# Autodesk Inventor assembly: Test Assembly
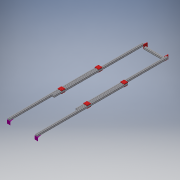
[picture p0: Inventor's stored thumbnail of the model, 180x180]
Saved by Autodesk Inventor 2016 SP2 (Build 200236200, 236)
## iProperties
Created: 2018-01-27
Part Number: Test Assembly
Document SubType Name: Assembly
Designer: CAD
Author: CAD
## Documents named in this file (5)
- C:\Users\CAD\Documents\GitHub\FIRST-ROBOTICS-2018-5436-CAD\Robot\Elevator\Test Assembly.iam
- C:\Users\CAD\Documents\GitHub\FIRST-ROBOTICS-2018-5436-CAD\Robot\Elevator\48 in 80-20 extrusion.ipt
- C:\Users\CAD\Documents\GitHub\FIRST-ROBOTICS-2018-5436-CAD\Robot\Elevator\80-20 extrusion rail.ipt
- C:\Users\CAD\Documents\GitHub\FIRST-ROBOTICS-2018-5436-CAD\Robot\Elevator\Bottom Elevator Bracket.ipt
- C:\Users\CAD\Documents\GitHub\FIRST-ROBOTICS-2018-5436-CAD\Robot\Elevator\10.75 in 80-20 extrusion.ipt
## Components (17 placed, 4 different names)
1. 48 in 80-20 extrusion:1 — Flush:1, Flush:3, Flush:5, Mate:16, Flush:12, Mate:26, Mate:27
2. 48 in 80-20 extrusion:2 — Flush:1, Mate:2, Mate:3, Mate:4, Mate:5, Flush:2, Mate:8, Mate:9, Mate:10, Mate:11, Flush:8, Flush:11, Mate:34, Mate:35, Angle:1
3. 48 in 80-20 extrusion:3 — Flush:5, Flush:6, Mate:19, Flush:11, Flush:13, Flush:14
4. 48 in 80-20 extrusion:4 — Flush:6, Mate:17, Mate:18, Mate:20, Mate:21, Flush:9, Flush:10, Flush:12, Mate:22, Mate:23, Mate:24, Mate:25, Mate:28, Mate:29, Flush:16
5. 80-20 extrusion rail:1 — Mate:2, Mate:3, Flush:2, Mate:6
6. 80-20 extrusion rail:2 — Mate:8, Mate:9, Flush:7, Mate:16
7. 80-20 extrusion rail:3 — Mate:10, Mate:11, Flush:8
8. 80-20 extrusion rail:4 — Mate:4, Mate:5, Flush:3, Mate:6, Flush:7
9. 80-20 extrusion rail:5 — Mate:17, Mate:18, Mate:19, Flush:9
10. 80-20 extrusion rail:8 — Mate:20, Mate:21, Flush:10
11. 80-20 extrusion rail:9 — Mate:24, Mate:25, Flush:14
12. 80-20 extrusion rail:10 — Mate:22, Mate:23, Flush:13
13. Bottom Elevator Bracket:1 — Mate:26, Mate:27, Flush:15
14. Bottom Elevator Bracket:2 — Mate:28, Mate:29, Flush:15, Flush:16
15. 10.75 in 80-20 extrusion:2 — Mate:32, Mate:33, Angle:1
16. 80-20 extrusion rail:11 — Flush:17, Flush:18
17. 80-20 extrusion rail:12 — Mate:32, Mate:33, Mate:34, Mate:35, Flush:17, Flush:18
## Relationships (45: Mate 27, Flush 17, Angle 1)
- Flush:1: 48 in 80-20 extrusion:1 ↔ 48 in 80-20 extrusion:2
- Mate:2: 48 in 80-20 extrusion:2 ↔ 80-20 extrusion rail:1
- Mate:3: 48 in 80-20 extrusion:2 ↔ 80-20 extrusion rail:1
- Mate:4: 48 in 80-20 extrusion:2 ↔ 80-20 extrusion rail:4
- Mate:5: 48 in 80-20 extrusion:2 ↔ 80-20 extrusion rail:4
- Flush:2 (101.6 mm): 48 in 80-20 extrusion:2 ↔ 80-20 extrusion rail:1
- Flush:3: 48 in 80-20 extrusion:1 ↔ 80-20 extrusion rail:4
- Mate:6 (136.7282 mm): 80-20 extrusion rail:1 ↔ 80-20 extrusion rail:4
- Flush:5: 48 in 80-20 extrusion:1 ↔ 48 in 80-20 extrusion:3
- Flush:6: 48 in 80-20 extrusion:3 ↔ 48 in 80-20 extrusion:4
- Mate:8: 48 in 80-20 extrusion:2 ↔ 80-20 extrusion rail:2
- Mate:9: 48 in 80-20 extrusion:2 ↔ 80-20 extrusion rail:2
- Flush:7: 80-20 extrusion rail:2 ↔ 80-20 extrusion rail:4
- Mate:10: 48 in 80-20 extrusion:2 ↔ 80-20 extrusion rail:3
- Mate:11: 48 in 80-20 extrusion:2 ↔ 80-20 extrusion rail:3
- Flush:8 (101.6 mm): 48 in 80-20 extrusion:2 ↔ 80-20 extrusion rail:3
- Mate:16: 48 in 80-20 extrusion:1 ↔ 80-20 extrusion rail:2
- Mate:17: 48 in 80-20 extrusion:4 ↔ 80-20 extrusion rail:5
- Mate:18: 48 in 80-20 extrusion:4 ↔ 80-20 extrusion rail:5
- Mate:19: 48 in 80-20 extrusion:3 ↔ 80-20 extrusion rail:5
- Mate:20: 48 in 80-20 extrusion:4 ↔ 80-20 extrusion rail:8
- Mate:21: 48 in 80-20 extrusion:4 ↔ 80-20 extrusion rail:8
- Flush:9: 48 in 80-20 extrusion:4 ↔ 80-20 extrusion rail:5
- Flush:10: 48 in 80-20 extrusion:4 ↔ 80-20 extrusion rail:8
- Flush:11: 48 in 80-20 extrusion:2 ↔ 48 in 80-20 extrusion:3
- Flush:12: 48 in 80-20 extrusion:1 ↔ 48 in 80-20 extrusion:4
- Mate:22: 48 in 80-20 extrusion:4 ↔ 80-20 extrusion rail:10
- Mate:23: 48 in 80-20 extrusion:4 ↔ 80-20 extrusion rail:10
- Flush:13 (101.6 mm): 48 in 80-20 extrusion:3 ↔ 80-20 extrusion rail:10
- Mate:24: 48 in 80-20 extrusion:4 ↔ 80-20 extrusion rail:9
- Mate:25: 48 in 80-20 extrusion:4 ↔ 80-20 extrusion rail:9
- Flush:14 (-101.6 mm): 48 in 80-20 extrusion:3 ↔ 80-20 extrusion rail:9
- Mate:26: 48 in 80-20 extrusion:1 ↔ Bottom Elevator Bracket:1
- Mate:27: 48 in 80-20 extrusion:1 ↔ Bottom Elevator Bracket:1
- Mate:28: 48 in 80-20 extrusion:4 ↔ Bottom Elevator Bracket:2
- Mate:29: 48 in 80-20 extrusion:4 ↔ Bottom Elevator Bracket:2
- Flush:15: Bottom Elevator Bracket:1 ↔ Bottom Elevator Bracket:2
- Flush:16: 48 in 80-20 extrusion:4 ↔ Bottom Elevator Bracket:2
- Mate:32: 10.75 in 80-20 extrusion:2 ↔ 80-20 extrusion rail:12
- Mate:33: 10.75 in 80-20 extrusion:2 ↔ 80-20 extrusion rail:12
- Mate:34: 48 in 80-20 extrusion:2 ↔ 80-20 extrusion rail:12
- Mate:35: 48 in 80-20 extrusion:2 ↔ 80-20 extrusion rail:12
- Flush:17: 80-20 extrusion rail:11 ↔ 80-20 extrusion rail:12
- Flush:18: 80-20 extrusion rail:11 ↔ 80-20 extrusion rail:12
- Angle:1 (0 deg): 48 in 80-20 extrusion:2 ↔ 10.75 in 80-20 extrusion:2
